# Autodesk Inventor assembly: hand_assembly
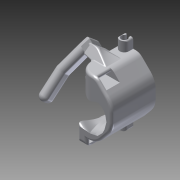
[picture p0: Inventor's stored thumbnail of the model, 180x180]
Saved by Autodesk Inventor 2015 (Build 190159000, 159)
## iProperties
Created: 2014-09-19
Part Number: hand_assembly
Document SubType Name: Assembly
Designer: Dale
Author: Dale
## Documents named in this file (3)
- C:\Users\Dale\Desktop\Split hand\Dale's updates\hand_assembly.iam
- C:\Users\Dale\Desktop\Split hand\Dale's updates\thumb2.ipt
- C:\Users\Dale\Desktop\Split hand\Dale's updates\new_palm.ipt
## Components (2 placed, 2 different names)
1. new_palm:1 — Mate:1, Mate:2
2. thumb2:1 — Mate:1, Mate:2
## Relationships (2: Mate 2)
- Mate:1: new_palm:1 ↔ thumb2:1
- Mate:2: new_palm:1 ↔ thumb2:1
